# Autodesk Inventor assembly: Final Assembly
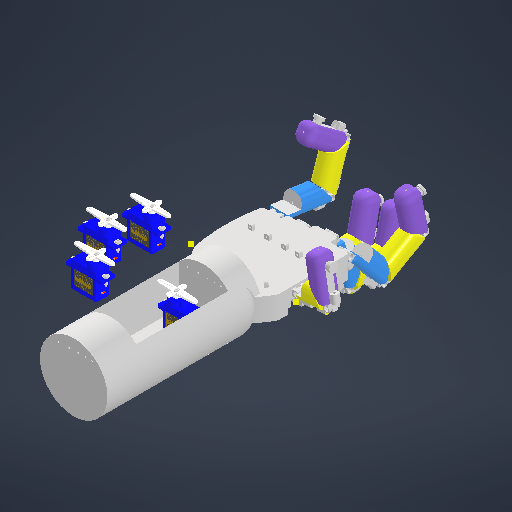
[picture p0: Inventor's stored thumbnail of the model, 512x512]
Saved by Autodesk Inventor 2026 (Build 300175050, 175E)
## iProperties
Created: 2026-05-23
Part Number: Final Assembly
Document SubType Name: Assembly
Designer: SaiAn
Author: SaiAn
## Documents named in this file (5)
- C:\EMG Biomechanical Arm\Final Assembly.iam
- C:\EMG Biomechanical Arm\Finger Assembly.iam
- C:\EMG Biomechanical Arm\Palm.ipt
- C:\Users\SaiAn\Downloads\SG90 - Micro Servo 9g - Tower Pro\SG90 - Micro Servo 9g - Tower Pro\SG90 - Micro Servo 9g - Tower Pro.ipt
- C:\EMG Biomechanical Arm\ThumbAssembly.iam
## Components (10 placed, 4 different names)
1. Finger Assembly:1 [sub-assembly] — Mate:1, Mate:2
2. Finger Assembly:2 [sub-assembly] — Mate:5, Mate:6
3. Finger Assembly:3 [sub-assembly] — Mate:7, Mate:8
4. Finger Assembly:4 [sub-assembly] — Mate:3, Mate:4
5. Palm:2 — Mate:1, Mate:2, Mate:3, Mate:4, Mate:5, Mate:6, Mate:7, Mate:8, Mate:9, Mate:10, Mate:11
6. SG90 - Micro Servo 9g - Tower Pro:1 — Mate:11
7. SG90 - Micro Servo 9g - Tower Pro:2
8. SG90 - Micro Servo 9g - Tower Pro:3
9. SG90 - Micro Servo 9g - Tower Pro:4
10. ThumbAssembly:1 [sub-assembly] — Mate:9, Mate:10
## Relationships (11: Mate 11)
- Mate:1: Finger Assembly:1 ↔ Palm:2
- Mate:2: Finger Assembly:1 ↔ Palm:2
- Mate:3: Finger Assembly:4 ↔ Palm:2
- Mate:4: Finger Assembly:4 ↔ Palm:2
- Mate:5: Finger Assembly:2 ↔ Palm:2
- Mate:6: Finger Assembly:2 ↔ Palm:2
- Mate:7: Finger Assembly:3 ↔ Palm:2
- Mate:8: Finger Assembly:3 ↔ Palm:2
- Mate:9: Palm:2 ↔ ThumbAssembly:1
- Mate:10: Palm:2 ↔ ThumbAssembly:1
- Mate:11: Palm:2 ↔ SG90 - Micro Servo 9g - Tower Pro:1
